# Autodesk Inventor assembly: DELL_DA-130PE1-00.ipt
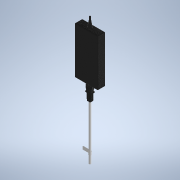
[picture p0: Inventor's stored thumbnail of the model, 180x180]
Saved by Autodesk Inventor 2021 (Build 250183000, 183)
## iProperties
Created: 2022-01-02
Part Number: DELL_DA-130PE1-00.ipt
Document SubType Name: Assembly
Designer: Jorian Brusind
Author: Jorian Brusind
## Documents named in this file (3)
- C:\Users\Jorian Brusind\Documents\GitHub\PersonalProjects\HyperRail\Inventor Files\DELL_DA-130PE1-00.ipt.iam
- C:\Users\Jorian Brusind\Documents\GitHub\PersonalProjects\HyperRail\Inventor Files\11-00055.iam
- C:\Users\Jorian Brusind\Documents\GitHub\PersonalProjects\HyperRail\Inventor Files\DELL_DA-130PE1-00_base.ipt
## Components (2 placed, 2 different names)
1. 11-00055:1 [sub-assembly] — Mate:1, Mate:2, Angle:1
2. DELL_DA-130PE1-00_base:1 — Mate:1, Mate:2, Angle:1
## Relationships (3: Mate 2, Angle 1)
- Mate:1: 11-00055:1 ↔ DELL_DA-130PE1-00_base:1
- Mate:2: 11-00055:1 ↔ DELL_DA-130PE1-00_base:1
- Angle:1 (90 deg): 11-00055:1 ↔ DELL_DA-130PE1-00_base:1
